# Autodesk Inventor assembly: Assembly2
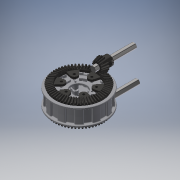
[picture p0: Inventor's stored thumbnail of the model, 180x180]
Saved by Autodesk Inventor 2019.3 (Build 233278000, 278)
## iProperties
Created: 2019-04-21
Part Number: Assembly2
Document SubType Name: Assembly
Designer: Connor
Author: Connor
## Documents named in this file (5)
- C:\Users\Connor\Documents\GrabCAD\NuSwerve\Assembly2.iam
- C:\Users\Connor\Documents\GrabCAD\NuSwerve\Imported Components\Wheels and Hubs\VEX Traction Wheels\TractionWheel 4x1\TractionWheel 4x1.iam
- C:\Users\Connor\Documents\GrabCAD\NuSwerve\15t_bevel.ipt
- C:\Users\Connor\Documents\GrabCAD\NuSwerve\60t_bevel.ipt
- C:\Users\Connor\Documents\GrabCAD\NuSwerve\drive_shaft.ipt
## Components (7 placed, 4 different names)
1. TractionWheel 4x1:1 [sub-assembly] — Mate:1, Mate:2, Mate:3, Mate:4, Mate:5, Mate:6
2. 15t_bevel:1 — Flush:2, Mate:7, Tangent:1, Mate:9, Mate:10
3. 60t_bevel:1 — Mate:1, Mate:2, Mate:3, Flush:2, Mate:7, Tangent:1
4. 15t_bevel:2 — Mate:8, Tangent:2, Flush:3, Mate:11, Mate:12
5. 60t_bevel:2 — Mate:4, Mate:5, Mate:6, Mate:8, Tangent:2, Flush:3
6. drive_shaft:1 — Mate:9, Mate:10
7. drive_shaft:2 — Mate:11, Mate:12
## Relationships (16: Mate 12, Flush 2, Tangent 2)
- Mate:1: TractionWheel 4x1:1 ↔ 60t_bevel:1
- Mate:2: TractionWheel 4x1:1 ↔ 60t_bevel:1
- Mate:3: TractionWheel 4x1:1 ↔ 60t_bevel:1
- Mate:4: TractionWheel 4x1:1 ↔ 60t_bevel:2
- Mate:5: TractionWheel 4x1:1 ↔ 60t_bevel:2
- Mate:6: TractionWheel 4x1:1 ↔ 60t_bevel:2
- Flush:2: 15t_bevel:1 ↔ 60t_bevel:1
- Mate:7 (-56 mm): 15t_bevel:1 ↔ 60t_bevel:1
- Tangent:1 (2 mm): 15t_bevel:1 ↔ 60t_bevel:1
- Mate:8: 15t_bevel:2 ↔ 60t_bevel:2
- Tangent:2 (2 mm): 15t_bevel:2 ↔ 60t_bevel:2
- Flush:3 (-56 mm): 15t_bevel:2 ↔ 60t_bevel:2
- Mate:9: 15t_bevel:1 ↔ drive_shaft:1
- Mate:10: 15t_bevel:1 ↔ drive_shaft:1
- Mate:11: 15t_bevel:2 ↔ drive_shaft:2
- Mate:12: 15t_bevel:2 ↔ drive_shaft:2
